# Autodesk Inventor assembly: ZAssembly
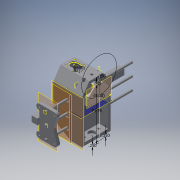
[picture p0: Inventor's stored thumbnail of the model, 180x180]
Saved by Autodesk Inventor 2016 (Build 200138000, 138)
## iProperties
Created: 2016-03-26
Part Number: ZAssembly
Document SubType Name: Assembly
Designer: Scott
Author: Scott
## Documents named in this file (6)
- C:\Users\Scott\Google Drive\Engineering Ideas and Designs\3D printer\Nefarian\ZAssembly.iam
- C:\Users\Scott\Google Drive\Engineering Ideas and Designs\3D printer\Nefarian\Z Nut.ipt
- C:\Users\Scott\Google Drive\Engineering Ideas and Designs\3D printer\Nefarian\ZFrame.ipt
- C:\Users\Scott\Google Drive\Engineering Ideas and Designs\3D printer\Nefarian\Z Slide.ipt
- C:\Users\Scott\Google Drive\Engineering Ideas and Designs\3D printer\Nefarian\Rails.ipt
- C:\Users\Scott\Google Drive\Engineering Ideas and Designs\3D printer\Nefarian\Endstop.ipt
## Components (5 placed, 5 different names)
1. Z Nut:1 — Flush:1, Flush:2, Flush:3, Flush:4, Flush:5
2. ZFrame:1 — Flush:1, Flush:2, Flush:3, Flush:4, Flush:5, Flush:6, Flush:7
3. Z Slide:1 — Flush:6, Flush:7, Flush:8, Flush:9, Flush:10
4. Rails:1 — Flush:9, Flush:10, Flush:11, Flush:12
5. Endstop:1 — Flush:11, Flush:12
## Relationships (12: Flush 12)
- Flush:1: Z Nut:1 ↔ ZFrame:1
- Flush:2: Z Nut:1 ↔ ZFrame:1
- Flush:3: Z Nut:1 ↔ ZFrame:1
- Flush:4 (3.175 mm): Z Nut:1 ↔ ZFrame:1
- Flush:5: Z Nut:1 ↔ ZFrame:1
- Flush:6: ZFrame:1 ↔ Z Slide:1
- Flush:7: ZFrame:1 ↔ Z Slide:1
- Flush:8 (49.2125 mm): Z Slide:1
- Flush:9: Z Slide:1 ↔ Rails:1
- Flush:10: Z Slide:1 ↔ Rails:1
- Flush:11: Rails:1 ↔ Endstop:1
- Flush:12 (-5.9944 mm): Rails:1 ↔ Endstop:1
